# Autodesk Inventor assembly: Unknown
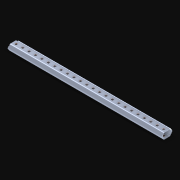
[picture p0: Inventor's stored thumbnail of the model, 180x180]
Saved by Autodesk Inventor 2021 (Build 250183000, 183)
## iProperties
Category: Motion
Company: Super Sonic Sparks, Team 24
Part Number: Unknown
Document SubType Name: Assembly
Designer: Jordan Kiesel
Mass: 175.632 g
Surface Area: 438.626 cm^2
Volume: 24.116 cm^3
Density: 7.28282 g/cm^3
Catalog Web Link: vexrobotics.com/276-1096.html
Description: The perfect solution for linear motion.
Vendor: VEX Robotics, Inc.
Created: 2020-06-02
Translation Standard: STEP AP203
FileName: Linear Slide Assembly.iam
PreProcessor: SolidWorks 2007
PostProcessor: Build: 239, Release: 2011 RTM - Date: Wed 02/17/2010
Sent Units: inch
Uncertainty: 1e-05
Author: Jordan Kiesel
Title: Linear Slide Assembly
Comments: The perfect solution for linear motion. The slides fit one inside the other. ▷ Each rail is 12" long. ▷ The rails have holes on 0.500" increments. ▷ Made from cold rolled steel, 0.046" thick, zinc plated.
## Documents named in this file (3)
- E:\2020 library 2\Motion\Linear Slide Assembly.iam
- E:\2020 library 2\Motion\Reference Parts\Linear Slide Assembly\Inner Slide Member.ipt
- E:\2020 library 2\Motion\Reference Parts\Linear Slide Assembly\Outer Slide Member.ipt
## Components (2 placed, 2 different names)
1. Outer Slide Member:1 — Flush:1, Mate:1
2. Inner Slide Member:1 — Flush:1, Mate:1
## Relationships (2: Flush 1, Mate 1)
- Flush:1: Outer Slide Member:1 ↔ Inner Slide Member:1
- Mate:1 (10.2108 mm): Outer Slide Member:1 ↔ Inner Slide Member:1
